# Autodesk Inventor assembly: instrumentBody
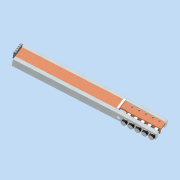
[picture p0: Inventor's stored thumbnail of the model, 180x180]
Saved by Autodesk Inventor 2021 (Build 250183000, 183)
## iProperties
Created: 2021-02-01
Part Number: instrumentBody
Document SubType Name: Assembly
Designer: garre
Author: garre
## Documents named in this file (8)
- C:\Users\garre\Desktop\Parts\instrumentBody.iam
- C:\Users\garre\Desktop\Parts\bodySidePlate.ipt
- C:\Users\garre\Desktop\Parts\bodyTopPlate.ipt
- C:\Users\garre\Desktop\Parts\bodyBotPlate.ipt
- C:\Users\garre\Desktop\Parts\LoadCell.ipt
- C:\Users\garre\Desktop\Parts\Nut.ipt
- C:\Users\garre\Desktop\Parts\TuningPeg.ipt
- C:\Users\garre\Desktop\Parts\MountedMotor.iam
## Components (20 placed, 7 different names)
1. bodySidePlate:1 — Mate:2, Flush:3, Flush:4, Mate:4, Mate:10, Mate:25
2. bodySidePlate:2 — Mate:1, Flush:1, Flush:2, Flush:5, Angle:1
3. bodyTopPlate:1 — Mate:1, Flush:1, Flush:2, Mate:2, Flush:3, Flush:4, Mate:5, Mate:6, Mate:7, Mate:8, Mate:9, Flush:6, Mate:11, Flush:15, Mate:12
4. bodyBotPlate:1 — Flush:5, Mate:4, Mate:13, Mate:14, Mate:15, Mate:16, Mate:17, Mate:18, Mate:19, Mate:20, Mate:21, Mate:22, Mate:25, Mate:26, Mate:27, Flush:16, Mate:28, Flush:17, Mate:30, Flush:18, Mate:32, Flush:19, Mate:34, Flush:20
5. LoadCell:1 — Mate:5, Flush:6, Flush:7, Flush:8, Flush:9, Flush:10, Flush:11, Flush:13
6. LoadCell:2 — Mate:6, Flush:10, Flush:11, Flush:12
7. LoadCell:3 — Mate:7, Flush:8, Flush:13
8. LoadCell:4 — Mate:8, Flush:7, Flush:12, Flush:14
9. LoadCell:5 — Mate:9, Flush:9, Flush:14, Mate:10
10. Nut:1 — Mate:11, Flush:15, Mate:12
11. TuningPeg:1 — Mate:13, Mate:18, Angle:1, Angle:2
12. TuningPeg:2 — Mate:14, Mate:20, Angle:3, Angle:4
13. TuningPeg:3 — Mate:16, Mate:19, Angle:2, Angle:3
14. TuningPeg:4 — Mate:17, Mate:22, Angle:5
15. TuningPeg:5 — Mate:15, Mate:21, Angle:4, Angle:5
16. MountedMotor:1 [sub-assembly] — Mate:26, Mate:27, Flush:16, Mate:29
17. MountedMotor:2 [sub-assembly] — Mate:28, Flush:17, Mate:29, Mate:31
18. MountedMotor:3 [sub-assembly] — Mate:30, Flush:18, Mate:31, Mate:33
19. MountedMotor:4 [sub-assembly] — Mate:32, Flush:19, Mate:33, Mate:35
20. MountedMotor:5 [sub-assembly] — Mate:34, Flush:20, Mate:35
## Relationships (57: Mate 32, Flush 20, Angle 5)
- Mate:1: bodySidePlate:2 ↔ bodyTopPlate:1
- Flush:1: bodySidePlate:2 ↔ bodyTopPlate:1
- Flush:2: bodySidePlate:2 ↔ bodyTopPlate:1
- Mate:2: bodySidePlate:1 ↔ bodyTopPlate:1
- Flush:3: bodySidePlate:1 ↔ bodyTopPlate:1
- Flush:4: bodySidePlate:1 ↔ bodyTopPlate:1
- Flush:5: bodySidePlate:2 ↔ bodyBotPlate:1
- Mate:4: bodySidePlate:1 ↔ bodyBotPlate:1
- Mate:5: bodyTopPlate:1 ↔ LoadCell:1
- Mate:6: bodyTopPlate:1 ↔ LoadCell:2
- Mate:7: bodyTopPlate:1 ↔ LoadCell:3
- Mate:8: bodyTopPlate:1 ↔ LoadCell:4
- Mate:9: bodyTopPlate:1 ↔ LoadCell:5
- Flush:6: bodyTopPlate:1 ↔ LoadCell:1
- Flush:7: LoadCell:1 ↔ LoadCell:4
- Flush:8: LoadCell:1 ↔ LoadCell:3
- Flush:9: LoadCell:1 ↔ LoadCell:5
- Flush:10: LoadCell:1 ↔ LoadCell:2
- Flush:11 (15.875 mm): LoadCell:1 ↔ LoadCell:2
- Flush:12 (15.875 mm): LoadCell:2 ↔ LoadCell:4
- Flush:13 (15.875 mm): LoadCell:1 ↔ LoadCell:3
- Flush:14 (-15.875 mm): LoadCell:4 ↔ LoadCell:5
- Mate:10: bodySidePlate:1 ↔ LoadCell:5
- Mate:11: bodyTopPlate:1 ↔ Nut:1
- Flush:15: bodyTopPlate:1 ↔ Nut:1
- Mate:12: bodyTopPlate:1 ↔ Nut:1
- Mate:13: bodyBotPlate:1 ↔ TuningPeg:1
- Mate:14: bodyBotPlate:1 ↔ TuningPeg:2
- Mate:15: bodyBotPlate:1 ↔ TuningPeg:5
- Mate:16: bodyBotPlate:1 ↔ TuningPeg:3
- Mate:17: bodyBotPlate:1 ↔ TuningPeg:4
- Mate:18: bodyBotPlate:1 ↔ TuningPeg:1
- Mate:19: bodyBotPlate:1 ↔ TuningPeg:3
- Mate:20: bodyBotPlate:1 ↔ TuningPeg:2
- Mate:21: bodyBotPlate:1 ↔ TuningPeg:5
- Mate:22: bodyBotPlate:1 ↔ TuningPeg:4
- Mate:25: bodySidePlate:1 ↔ bodyBotPlate:1
- Mate:26: bodyBotPlate:1 ↔ MountedMotor:1
- Mate:27: bodyBotPlate:1 ↔ MountedMotor:1
- Angle:1 (180 deg): bodySidePlate:2 ↔ TuningPeg:1
- Flush:16: bodyBotPlate:1 ↔ MountedMotor:1
- Mate:28: bodyBotPlate:1 ↔ MountedMotor:2
- Flush:17: bodyBotPlate:1 ↔ MountedMotor:2
- Mate:29: MountedMotor:1 ↔ MountedMotor:2
- Angle:2 (0 deg): TuningPeg:1 ↔ TuningPeg:3
- Angle:3 (0 deg): TuningPeg:2 ↔ TuningPeg:3
- Angle:4 (0 deg): TuningPeg:2 ↔ TuningPeg:5
- Angle:5 (0 deg): TuningPeg:4 ↔ TuningPeg:5
- Mate:30: bodyBotPlate:1 ↔ MountedMotor:3
- Flush:18: bodyBotPlate:1 ↔ MountedMotor:3
- Mate:31: MountedMotor:2 ↔ MountedMotor:3
- Mate:32: bodyBotPlate:1 ↔ MountedMotor:4
- Flush:19: bodyBotPlate:1 ↔ MountedMotor:4
- Mate:33: MountedMotor:3 ↔ MountedMotor:4
- Mate:34: bodyBotPlate:1 ↔ MountedMotor:5
- Flush:20: bodyBotPlate:1 ↔ MountedMotor:5
- Mate:35: MountedMotor:4 ↔ MountedMotor:5
## Named parameters: loadCellWidth = 0 mm, stringSeparation = 12.7 mm, stringHorizontalOffset = 0 mm, loadCellSeparation = 3.175 mm, motorSeparation = 0 mm
